# Autodesk Inventor assembly: Riel50CM_completo
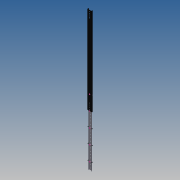
[picture p0: Inventor's stored thumbnail of the model, 180x180]
Saved by Autodesk Inventor 2011 (Build 150239000, 239)
## iProperties
Created: 2011-09-24
Part Number: Riel50CM_completo
Document SubType Name: Assembly
Designer: mgaspari
Author: mgaspari
## Documents named in this file (3)
- C:\Users\IBM_ADMIN\Desktop\cilindro\Mio\Guia\Riel50CM_completo.iam
- C:\Users\IBM_ADMIN\Desktop\cilindro\Mio\Guia\riel.ipt
- C:\Users\IBM_ADMIN\Desktop\cilindro\Mio\Guia\trencompleto.iam
## Components (2 placed, 2 different names)
1. riel:1 — Tangent:1, Mate:1
2. trencompleto:1 [sub-assembly] — Tangent:1, Mate:1
## Relationships (2: Tangent 1, Mate 1)
- Tangent:1: riel:1 ↔ trencompleto:1
- Mate:1 (400 mm): riel:1 ↔ trencompleto:1
